# Autodesk Inventor assembly: INDX_000_Shuffler
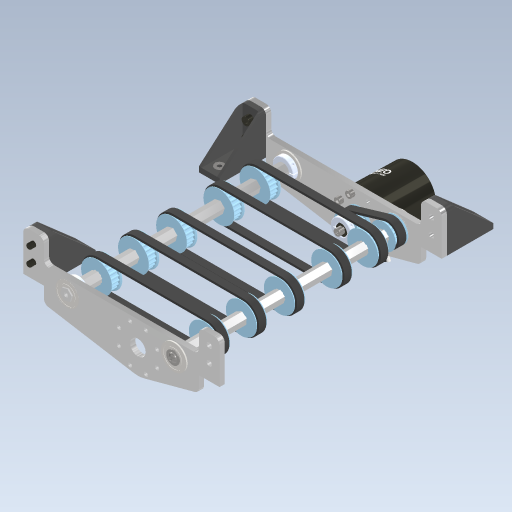
[picture p0: Inventor's stored thumbnail of the model, 512x512]
Saved by Autodesk Inventor 2024 (Build 280153000, 153)
## iProperties
Created: 2024-08-08
Part Number: INDX_000_Shuffler
Document SubType Name: Assembly
Designer: Oscar
Author: Oscar
## Documents named in this file (19)
- C:\Users\Takum\OneDrive\Documents\GitHub\1622-2024-Summer-CAD-A-Thon\Index\INDX_000_Shuffler.iam
- C:\Users\Takum\OneDrive\Documents\GitHub\1622-2024-Summer-CAD-A-Thon\Index\INDX_004_shufflePlate.ipt
- C:\Users\Takum\OneDrive\Documents\GitHub\1622-2024-Summer-CAD-A-Thon\Drive Base\DVBS_001_Full Assembly.iam
- C:\Users\Takum\OneDrive\Documents\GitHub\1622-2024-Summer-CAD-A-Thon\Index\INDX_005_Cornerbracket.ipt
- C:\Users\Takum\OneDrive\Documents\GitHub\1622-2024-Summer-CAD-A-Thon\COTS Library\Motors\COTS_REV-21-1650-V1.1_Neo1.1.ipt
- C:\Users\Takum\OneDrive\Documents\GitHub\1622-2024-Summer-CAD-A-Thon\COTS Library\Motion\Bearings\COTS_WCP-0783_1.125ODHexBearing.ipt
- C:\Users\Takum\OneDrive\Documents\GitHub\1622-2024-Summer-CAD-A-Thon\COTS Library\Structural Adapter\COTS_WCP-0794_0.5inshaftadapter.ipt
- C:\Users\Takum\OneDrive\Documents\GitHub\1622-2024-Summer-CAD-A-Thon\Index\INDX_018_FeederHex.ipt
- C:\Users\Takum\OneDrive\Documents\GitHub\1622-2024-Summer-CAD-A-Thon\COTS Library\Motion\Pulleys\HTD5M\10mm Wide\COTS_HTD5MM_9mm_16TPulley.ipt
- C:\Users\Takum\OneDrive\Documents\GitHub\1622-2024-Summer-CAD-A-Thon\Index\INDX_013_ThinSpacer.ipt
- C:\Users\Takum\OneDrive\Documents\GitHub\1622-2024-Summer-CAD-A-Thon\Index\INDX_007_22TPulley.ipt
- C:\Users\Takum\OneDrive\Documents\GitHub\1622-2024-Summer-CAD-A-Thon\COTS Library\Fasteners\Shaft Collars\COTS_WCP-0799_0.5inchHexShaftCollar.ipt
- C:\Users\Takum\OneDrive\Documents\GitHub\1622-2024-Summer-CAD-A-Thon\Index\INDX_019_FeederBelt.ipt
- C:\Users\Takum\OneDrive\Documents\GitHub\1622-2024-Summer-CAD-A-Thon\Index\INDX_020_MiniFeederBelt.ipt
- C:\Users\Takum\OneDrive\Documents\GitHub\1622-2024-Summer-CAD-A-Thon\COTS Library\Fasteners\Washers\COTS_90107A029_316 Stainless Steel Washer.ipt
- C:\Users\Takum\OneDrive\Documents\GitHub\1622-2024-Summer-CAD-A-Thon\COTS Library\Fasteners\Washers\COTS_91860A047_Size10Washer.ipt
- C:\Users\Takum\OneDrive\Documents\GitHub\1622-2024-Summer-CAD-A-Thon\COTS Library\Fasteners\Bolts\Button-Head\0.25-20\COTS_0.25-20_ButtonHead_0.5inlong_StainlessSteel_92949A537.ipt
- C:\Users\Takum\OneDrive\Documents\GitHub\1622-2024-Summer-CAD-A-Thon\COTS Library\Fasteners\Bolts\Socket-Head\10-32\COTS_91251A340__3-18in long_Black-Oxide Alloy Steel Socket Head.ipt
- C:\Users\Takum\OneDrive\Documents\GitHub\1622-2024-Summer-CAD-A-Thon\COTS Library\Fasteners\Bolts\Socket-Head\0.25-20\COTS_91251A540_Black-Oxide Alloy Steel Socket Head Screw.ipt
## Components (52 placed, 18 different names)
1. INDX_004_shufflePlate:1 — Mate:9, Mate:10, Mate:11, Mate:34, Mate:35, Mate:36, Mate:37
2. INDX_004_shufflePlate:2 — Mate:4, Mate:5, Mate:6, Mate:7, Mate:22, Mate:24, Mate:25, Mate:26, Mate:27, Mate:28, Mate:31, Mate:32, Mate:33, Mate:40, Mate:97, Mate:98, Mate:99, Mate:100, Mate:101, Mate:102, Mate:103, Mate:104
3. DVBS_001_Full Assembly:1 [sub-assembly] — Mate:4, Mate:8, Mate:12, Mate:16, Mate:17, Mate:18
4. INDX_005_Cornerbracket:1 — Mate:9, Mate:10, Mate:11, Mate:12, Mate:17, Mate:18, Mate:84, Mate:85, Mate:86, Mate:87, Mate:109, Mate:110, Mate:111, Mate:112
5. INDX_005_Cornerbracket:2 — Mate:5, Mate:6, Mate:7, Mate:8, Mate:16, Mate:88, Mate:89, Mate:90, Mate:91, Mate:105, Mate:106, Mate:107, Mate:108
6. COTS_REV-21-1650-V1.1_Neo1.1:1 — Mate:22, Mate:24, Mate:29, Mate:30, Mate:40, Mate:41, Mate:60
7. COTS_WCP-0783_1.125ODHexBearing:1 — Mate:25, Mate:26, Mate:58, Mate:59
8. COTS_WCP-0783_1.125ODHexBearing:2 — Mate:27, Mate:28, Mate:42, Mate:43, Mate:44, Mate:82, Mate:83
9. COTS_WCP-0794_0.5inshaftadapter:1 — Mate:29, Mate:30
10. INDX_005_Cornerbracket:3 — Mate:31, Mate:32, Mate:33
11. COTS_WCP-0783_1.125ODHexBearing:3 — Mate:34, Mate:35, Mate:39, Flush:2, Mate:47, Mate:49, Mate:51, Mate:53, Mate:55, Mate:56, Mate:57
12. COTS_WCP-0783_1.125ODHexBearing:5 — Mate:36, Mate:37, Mate:38, Flush:1, Mate:46, Mate:48, Mate:50, Mate:52, Mate:54, Mate:80
13. INDX_018_FeederHex:1 — Mate:39, Flush:2
14. INDX_018_FeederHex:2 — Mate:38, Flush:1, Mate:81, Mate:92, Mate:94
15. COTS_HTD5MM_9mm_16TPulley:1 — Mate:41, Flush:3, Mate:61, Mate:77
16. COTS_HTD5MM_9mm_16TPulley:2 — Mate:42, Flush:3, Mate:45, Mate:78, Mate:79
17. INDX_013_ThinSpacer:1 — Mate:43, Mate:44, Mate:45
18. INDX_007_22TPulley:1 — Mate:46, Flush:4, Mate:62
19. INDX_007_22TPulley:2 — Mate:47, Flush:4, Mate:63, Mate:64
20. INDX_007_22TPulley:3 — Mate:49, Flush:5, Mate:66, Mate:67
21. INDX_007_22TPulley:4 — Mate:48, Flush:5, Mate:65
22. INDX_007_22TPulley:5 — Mate:50, Flush:6, Mate:72, Mate:73
23. INDX_007_22TPulley:6 — Mate:51, Flush:6, Mate:71
24. INDX_007_22TPulley:7 — Mate:52, Flush:7, Mate:76
25. INDX_007_22TPulley:8 — Mate:53, Flush:7, Mate:74, Mate:75
26. INDX_007_22TPulley:9 — Mate:55, Flush:8, Mate:69, Mate:70
27. INDX_007_22TPulley:10 — Mate:54, Flush:8, Mate:68
28. COTS_WCP-0799_0.5inchHexShaftCollar:1 — Mate:58, Mate:59
29. COTS_WCP-0799_0.5inchHexShaftCollar:2 — Mate:56, Mate:57
30. COTS_WCP-0799_0.5inchHexShaftCollar:3 — Mate:60, Mate:61
31. INDX_019_FeederBelt:1 — Mate:62, Mate:63, Mate:64
32. INDX_019_FeederBelt:2 — Mate:65, Mate:66, Mate:67
33. INDX_019_FeederBelt:3 — Mate:68, Mate:69, Mate:70
34. INDX_019_FeederBelt:4 — Mate:71, Mate:72, Mate:73
35. INDX_019_FeederBelt:5 — Mate:74, Mate:75, Mate:76
36. INDX_020_MiniFeederBelt:1 — Mate:77, Mate:78, Mate:79
37. COTS_90107A029_316 Stainless Steel Washer:1 — Mate:80, Mate:81, Mate:93
38. COTS_90107A029_316 Stainless Steel Washer:2 — Mate:82, Mate:83, Mate:95
39. COTS_91860A047_Size10Washer:1 — Mate:86, Mate:87
40. COTS_91860A047_Size10Washer:2 — Mate:90, Mate:91
41. COTS_91860A047_Size10Washer:3 — Mate:84, Mate:85
42. COTS_91860A047_Size10Washer:4 — Mate:88, Mate:89
43. COTS_0.25-20_ButtonHead_0.5inlong_StainlessSteel_92949A537:1 — Mate:92, Mate:93
44. COTS_0.25-20_ButtonHead_0.5inlong_StainlessSteel_92949A537:2 — Mate:94, Mate:95
45. COTS_91251A340__3-18in long_Black-Oxide Alloy Steel Socket Head:2 — Mate:97, Mate:101
46. COTS_91251A340__3-18in long_Black-Oxide Alloy Steel Socket Head:3 — Mate:98, Mate:102
47. COTS_91251A340__3-18in long_Black-Oxide Alloy Steel Socket Head:4 — Mate:100, Mate:104
48. COTS_91251A340__3-18in long_Black-Oxide Alloy Steel Socket Head:5 — Mate:99, Mate:103
49. COTS_91251A540_Black-Oxide Alloy Steel Socket Head Screw:1 — Mate:105, Mate:107
50. COTS_91251A540_Black-Oxide Alloy Steel Socket Head Screw:2 — Mate:106, Mate:108
51. COTS_91251A540_Black-Oxide Alloy Steel Socket Head Screw:3 — Mate:109, Mate:111
52. COTS_91251A540_Black-Oxide Alloy Steel Socket Head Screw:4 — Mate:110, Mate:112
## Relationships (109: Mate 101, Flush 8)
- Mate:4: INDX_004_shufflePlate:2 ↔ DVBS_001_Full Assembly:1
- Mate:5: INDX_004_shufflePlate:2 ↔ INDX_005_Cornerbracket:2
- Mate:6: INDX_004_shufflePlate:2 ↔ INDX_005_Cornerbracket:2
- Mate:7: INDX_004_shufflePlate:2 ↔ INDX_005_Cornerbracket:2
- Mate:8: DVBS_001_Full Assembly:1 ↔ INDX_005_Cornerbracket:2
- Mate:9: INDX_004_shufflePlate:1 ↔ INDX_005_Cornerbracket:1
- Mate:10: INDX_004_shufflePlate:1 ↔ INDX_005_Cornerbracket:1
- Mate:11: INDX_004_shufflePlate:1 ↔ INDX_005_Cornerbracket:1
- Mate:12: DVBS_001_Full Assembly:1 ↔ INDX_005_Cornerbracket:1
- Mate:16: DVBS_001_Full Assembly:1 ↔ INDX_005_Cornerbracket:2
- Mate:17: DVBS_001_Full Assembly:1 ↔ INDX_005_Cornerbracket:1
- Mate:18: DVBS_001_Full Assembly:1 ↔ INDX_005_Cornerbracket:1
- Mate:22: INDX_004_shufflePlate:2 ↔ COTS_REV-21-1650-V1.1_Neo1.1:1
- Mate:24: INDX_004_shufflePlate:2 ↔ COTS_REV-21-1650-V1.1_Neo1.1:1
- Mate:25: INDX_004_shufflePlate:2 ↔ COTS_WCP-0783_1.125ODHexBearing:1
- Mate:26: INDX_004_shufflePlate:2 ↔ COTS_WCP-0783_1.125ODHexBearing:1
- Mate:27: INDX_004_shufflePlate:2 ↔ COTS_WCP-0783_1.125ODHexBearing:2
- Mate:28: INDX_004_shufflePlate:2 ↔ COTS_WCP-0783_1.125ODHexBearing:2
- Mate:29: COTS_REV-21-1650-V1.1_Neo1.1:1 ↔ COTS_WCP-0794_0.5inshaftadapter:1
- Mate:30: COTS_REV-21-1650-V1.1_Neo1.1:1 ↔ COTS_WCP-0794_0.5inshaftadapter:1
- Mate:31: INDX_004_shufflePlate:2 ↔ INDX_005_Cornerbracket:3
- Mate:32: INDX_004_shufflePlate:2 ↔ INDX_005_Cornerbracket:3
- Mate:33: INDX_004_shufflePlate:2 ↔ INDX_005_Cornerbracket:3
- Mate:34: INDX_004_shufflePlate:1 ↔ COTS_WCP-0783_1.125ODHexBearing:3
- Mate:35: INDX_004_shufflePlate:1 ↔ COTS_WCP-0783_1.125ODHexBearing:3
- Mate:36: INDX_004_shufflePlate:1 ↔ COTS_WCP-0783_1.125ODHexBearing:5
- Mate:37: INDX_004_shufflePlate:1 ↔ COTS_WCP-0783_1.125ODHexBearing:5
- Mate:38: COTS_WCP-0783_1.125ODHexBearing:5 ↔ INDX_018_FeederHex:2
- Flush:1: COTS_WCP-0783_1.125ODHexBearing:5 ↔ INDX_018_FeederHex:2
- Mate:39: COTS_WCP-0783_1.125ODHexBearing:3 ↔ INDX_018_FeederHex:1
- Flush:2 (-1.5875 mm): COTS_WCP-0783_1.125ODHexBearing:3 ↔ INDX_018_FeederHex:1
- Mate:40: INDX_004_shufflePlate:2 ↔ COTS_REV-21-1650-V1.1_Neo1.1:1
- Mate:41: COTS_REV-21-1650-V1.1_Neo1.1:1 ↔ COTS_HTD5MM_9mm_16TPulley:1
- Mate:42: COTS_WCP-0783_1.125ODHexBearing:2 ↔ COTS_HTD5MM_9mm_16TPulley:2
- Flush:3: COTS_HTD5MM_9mm_16TPulley:1 ↔ COTS_HTD5MM_9mm_16TPulley:2
- Mate:43: COTS_WCP-0783_1.125ODHexBearing:2 ↔ INDX_013_ThinSpacer:1
- Mate:44: COTS_WCP-0783_1.125ODHexBearing:2 ↔ INDX_013_ThinSpacer:1
- Mate:45: COTS_HTD5MM_9mm_16TPulley:2 ↔ INDX_013_ThinSpacer:1
- Mate:46: COTS_WCP-0783_1.125ODHexBearing:5 ↔ INDX_007_22TPulley:1
- Mate:47: COTS_WCP-0783_1.125ODHexBearing:3 ↔ INDX_007_22TPulley:2
- Flush:4: INDX_007_22TPulley:1 ↔ INDX_007_22TPulley:2
- Mate:48: COTS_WCP-0783_1.125ODHexBearing:5 ↔ INDX_007_22TPulley:4
- Mate:49: COTS_WCP-0783_1.125ODHexBearing:3 ↔ INDX_007_22TPulley:3
- Flush:5: INDX_007_22TPulley:3 ↔ INDX_007_22TPulley:4
- Mate:50: COTS_WCP-0783_1.125ODHexBearing:5 ↔ INDX_007_22TPulley:5
- Mate:51: COTS_WCP-0783_1.125ODHexBearing:3 ↔ INDX_007_22TPulley:6
- Flush:6: INDX_007_22TPulley:5 ↔ INDX_007_22TPulley:6
- Mate:52: COTS_WCP-0783_1.125ODHexBearing:5 ↔ INDX_007_22TPulley:7
- Mate:53: COTS_WCP-0783_1.125ODHexBearing:3 ↔ INDX_007_22TPulley:8
- Flush:7: INDX_007_22TPulley:7 ↔ INDX_007_22TPulley:8
- Mate:54: COTS_WCP-0783_1.125ODHexBearing:5 ↔ INDX_007_22TPulley:10
- Mate:55: COTS_WCP-0783_1.125ODHexBearing:3 ↔ INDX_007_22TPulley:9
- Flush:8: INDX_007_22TPulley:9 ↔ INDX_007_22TPulley:10
- Mate:56: COTS_WCP-0783_1.125ODHexBearing:3 ↔ COTS_WCP-0799_0.5inchHexShaftCollar:2
- Mate:57: COTS_WCP-0783_1.125ODHexBearing:3 ↔ COTS_WCP-0799_0.5inchHexShaftCollar:2
- Mate:58: COTS_WCP-0783_1.125ODHexBearing:1 ↔ COTS_WCP-0799_0.5inchHexShaftCollar:1
- Mate:59: COTS_WCP-0783_1.125ODHexBearing:1 ↔ COTS_WCP-0799_0.5inchHexShaftCollar:1
- Mate:60: COTS_REV-21-1650-V1.1_Neo1.1:1 ↔ COTS_WCP-0799_0.5inchHexShaftCollar:3
- Mate:61: COTS_HTD5MM_9mm_16TPulley:1 ↔ COTS_WCP-0799_0.5inchHexShaftCollar:3
- Mate:62: INDX_007_22TPulley:1 ↔ INDX_019_FeederBelt:1
- Mate:63: INDX_007_22TPulley:2 ↔ INDX_019_FeederBelt:1
- Mate:64: INDX_007_22TPulley:2 ↔ INDX_019_FeederBelt:1
- Mate:65: INDX_007_22TPulley:4 ↔ INDX_019_FeederBelt:2
- Mate:66: INDX_007_22TPulley:3 ↔ INDX_019_FeederBelt:2
- Mate:67 (0.5 mm): INDX_007_22TPulley:3 ↔ INDX_019_FeederBelt:2
- Mate:68: INDX_007_22TPulley:10 ↔ INDX_019_FeederBelt:3
- Mate:69: INDX_007_22TPulley:9 ↔ INDX_019_FeederBelt:3
- Mate:70 (0.5 mm): INDX_007_22TPulley:9 ↔ INDX_019_FeederBelt:3
- Mate:71: INDX_007_22TPulley:6 ↔ INDX_019_FeederBelt:4
- Mate:72: INDX_007_22TPulley:5 ↔ INDX_019_FeederBelt:4
- Mate:73 (0.5 mm): INDX_007_22TPulley:5 ↔ INDX_019_FeederBelt:4
- Mate:74: INDX_007_22TPulley:8 ↔ INDX_019_FeederBelt:5
- Mate:75 (0.5 mm): INDX_007_22TPulley:8 ↔ INDX_019_FeederBelt:5
- Mate:76: INDX_007_22TPulley:7 ↔ INDX_019_FeederBelt:5
- Mate:77: COTS_HTD5MM_9mm_16TPulley:1 ↔ INDX_020_MiniFeederBelt:1
- Mate:78: COTS_HTD5MM_9mm_16TPulley:2 ↔ INDX_020_MiniFeederBelt:1
- Mate:79 (0.5 mm): COTS_HTD5MM_9mm_16TPulley:2 ↔ INDX_020_MiniFeederBelt:1
- Mate:80: COTS_WCP-0783_1.125ODHexBearing:5 ↔ COTS_90107A029_316 Stainless Steel Washer:1
- Mate:81: INDX_018_FeederHex:2 ↔ COTS_90107A029_316 Stainless Steel Washer:1
- Mate:82: COTS_WCP-0783_1.125ODHexBearing:2 ↔ COTS_90107A029_316 Stainless Steel Washer:2
- Mate:83: COTS_WCP-0783_1.125ODHexBearing:2 ↔ COTS_90107A029_316 Stainless Steel Washer:2
- Mate:84: INDX_005_Cornerbracket:1 ↔ COTS_91860A047_Size10Washer:3
- Mate:85: INDX_005_Cornerbracket:1 ↔ COTS_91860A047_Size10Washer:3
- Mate:86: INDX_005_Cornerbracket:1 ↔ COTS_91860A047_Size10Washer:1
- Mate:87: INDX_005_Cornerbracket:1 ↔ COTS_91860A047_Size10Washer:1
- Mate:88: INDX_005_Cornerbracket:2 ↔ COTS_91860A047_Size10Washer:4
- Mate:89: INDX_005_Cornerbracket:2 ↔ COTS_91860A047_Size10Washer:4
- Mate:90: INDX_005_Cornerbracket:2 ↔ COTS_91860A047_Size10Washer:2
- Mate:91: INDX_005_Cornerbracket:2 ↔ COTS_91860A047_Size10Washer:2
- Mate:92: INDX_018_FeederHex:2 ↔ COTS_0.25-20_ButtonHead_0.5inlong_StainlessSteel_92949A537:1
- Mate:93: COTS_90107A029_316 Stainless Steel Washer:1 ↔ COTS_0.25-20_ButtonHead_0.5inlong_StainlessSteel_92949A537:1
- Mate:94: INDX_018_FeederHex:2 ↔ COTS_0.25-20_ButtonHead_0.5inlong_StainlessSteel_92949A537:2
- Mate:95: COTS_90107A029_316 Stainless Steel Washer:2 ↔ COTS_0.25-20_ButtonHead_0.5inlong_StainlessSteel_92949A537:2
- Mate:97: INDX_004_shufflePlate:2 ↔ COTS_91251A340__3-18in long_Black-Oxide Alloy Steel Socket Head:2
- Mate:98: INDX_004_shufflePlate:2 ↔ COTS_91251A340__3-18in long_Black-Oxide Alloy Steel Socket Head:3
- Mate:99: INDX_004_shufflePlate:2 ↔ COTS_91251A340__3-18in long_Black-Oxide Alloy Steel Socket Head:5
- Mate:100: INDX_004_shufflePlate:2 ↔ COTS_91251A340__3-18in long_Black-Oxide Alloy Steel Socket Head:4
- Mate:101: INDX_004_shufflePlate:2 ↔ COTS_91251A340__3-18in long_Black-Oxide Alloy Steel Socket Head:2
- Mate:102: INDX_004_shufflePlate:2 ↔ COTS_91251A340__3-18in long_Black-Oxide Alloy Steel Socket Head:3
- Mate:103: INDX_004_shufflePlate:2 ↔ COTS_91251A340__3-18in long_Black-Oxide Alloy Steel Socket Head:5
- Mate:104: INDX_004_shufflePlate:2 ↔ COTS_91251A340__3-18in long_Black-Oxide Alloy Steel Socket Head:4
- Mate:105: INDX_005_Cornerbracket:2 ↔ COTS_91251A540_Black-Oxide Alloy Steel Socket Head Screw:1
- Mate:106: INDX_005_Cornerbracket:2 ↔ COTS_91251A540_Black-Oxide Alloy Steel Socket Head Screw:2
- Mate:107: INDX_005_Cornerbracket:2 ↔ COTS_91251A540_Black-Oxide Alloy Steel Socket Head Screw:1
- Mate:108: INDX_005_Cornerbracket:2 ↔ COTS_91251A540_Black-Oxide Alloy Steel Socket Head Screw:2
- Mate:109: INDX_005_Cornerbracket:1 ↔ COTS_91251A540_Black-Oxide Alloy Steel Socket Head Screw:3
- Mate:110: INDX_005_Cornerbracket:1 ↔ COTS_91251A540_Black-Oxide Alloy Steel Socket Head Screw:4
- Mate:111: INDX_005_Cornerbracket:1 ↔ COTS_91251A540_Black-Oxide Alloy Steel Socket Head Screw:3
- Mate:112: INDX_005_Cornerbracket:1 ↔ COTS_91251A540_Black-Oxide Alloy Steel Socket Head Screw:4
